# Autodesk Inventor assembly: MARS Micromouse Box
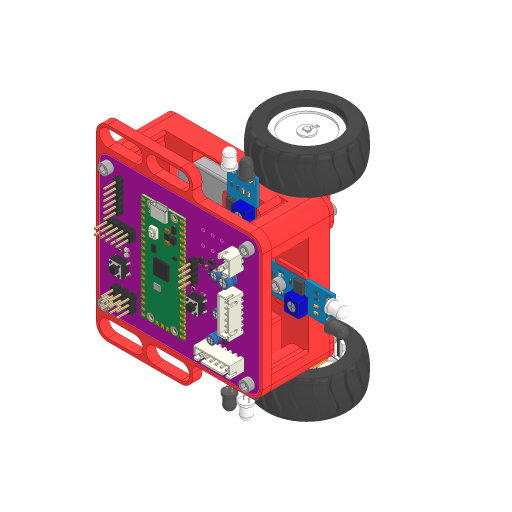
[picture p0: Inventor's stored thumbnail of the model, 512x512]
Saved by Autodesk Inventor 2024 (Build 280153000, 153)
## iProperties
Created: 2026-07-12
Part Number: MARS Micromouse Box
Document SubType Name: Assembly
Designer: Binara
Title: MARS Micromouse.step
Sending System: Autodesk Translation Framework v15.8.0.0
Preprocessor: ST-DEVELOPER v20.1
## Documents named in this file (12)
- Z:\Robotics\MARS\Micromouse Robot\starter-micromouse\CAD\MARS Micromouse\MARS Micromouse.iam
- Z:\Robotics\MARS\Micromouse Robot\starter-micromouse\CAD\MARS Micromouse\MARS_Micromouse_PCB v1.iam
- Z:\Robotics\MARS\Micromouse Robot\starter-micromouse\CAD\MARS Micromouse\Top Plate.ipt
- Z:\Robotics\MARS\Micromouse Robot\starter-micromouse\CAD\MARS Micromouse\Base Plate.ipt
- Z:\Robotics\MARS\Micromouse Robot\starter-micromouse\CAD\MARS Micromouse\IR_Sensor_YL63 v1.ipt
- Z:\Robotics\MARS\Micromouse Robot\starter-micromouse\CAD\MARS Micromouse\N20 Mini Micro Metall Gear Motor v1.ipt
- Z:\Robotics\MARS\Micromouse Robot\starter-micromouse\CAD\MARS Micromouse\RC wheel v1.iam
- Z:\Robotics\MARS\Micromouse Robot\starter-micromouse\CAD\MARS Micromouse\Motor Clamp.ipt
- Z:\Robotics\MARS\Micromouse Robot\starter-micromouse\CAD\MARS Micromouse\Caster Ball Extension.ipt
- Z:\Robotics\MARS\Micromouse Robot\starter-micromouse\CAD\MARS Micromouse\Caster Ball v3.ipt
- Z:\Robotics\MARS\Micromouse Robot\starter-micromouse\CAD\MARS Micromouse\New Battery.ipt
- Z:\Robotics\Inventor\Hardware\M3 x 8 screw\M3 x 8 screw.ipt
## Components (30 placed, 11 different names)
1. MARS_Micromouse_PCB v1:1 [sub-assembly] — Rigid:2, Cylindrical:1, Cylindrical:2, Rigid:3
2. Top Plate:1
3. Base Plate:1
4. IR_Sensor_YL63 v1:1 — Rotational:8
5. IR_Sensor_YL63 v1:2 — Rotational:9
6. IR_Sensor_YL63 v1:3 — Rotational:10
7. N20 Mini Micro Metall Gear Motor v1:1
8. N20 Mini Micro Metall Gear Motor v1:2
9. RC wheel v1:1 [sub-assembly]
10. RC wheel v1:2 [sub-assembly]
11. Motor Clamp:1 — Rotational:2, Rotational:3
12. Motor Clamp:2 — Rotational:4, Rotational:5
13. Caster Ball Extension:1 — Rotational:6, Rotational:7
14. Caster Ball v3:1 — Rigid:1, Rotational:1
15. New Battery:1
16. M3 x 8 screw:1 — Rotational:8
17. M3 x 8 screw:2 — Rigid:2
18. M3 x 8 screw:3 — Cylindrical:2
19. M3 x 8 screw:4 — Rigid:3
20. M3 x 8 screw:5 — Cylindrical:1
21. M3 x 8 screw:6 — Rotational:7
22. M3 x 8 screw:7 — Rotational:2
23. M3 x 8 screw:8 — Rotational:3
24. M3 x 8 screw:9 — Rotational:4
25. M3 x 8 screw:10 — Rotational:5
26. M3 x 8 screw:11 — Rotational:6
27. M3 x 8 screw:12 — Rigid:1
28. M3 x 8 screw:13 — Rotational:1
29. M3 x 8 screw:14 — Rotational:9
30. M3 x 8 screw:15 — Rotational:10
## Relationships (15: RevoluteJoint 10, WeldJoint 3, CylindricalJoint 2)
- Rigid:1 [WeldJoint]: Caster Ball v3:1 ↔ M3 x 8 screw:12
- Rotational:1 [RevoluteJoint]: Caster Ball v3:1 ↔ M3 x 8 screw:13
- Rotational:2 [RevoluteJoint]: Motor Clamp:1 ↔ M3 x 8 screw:7
- Rotational:3 [RevoluteJoint]: Motor Clamp:1 ↔ M3 x 8 screw:8
- Rotational:4 [RevoluteJoint]: Motor Clamp:2 ↔ M3 x 8 screw:9
- Rotational:5 [RevoluteJoint]: Motor Clamp:2 ↔ M3 x 8 screw:10
- Rotational:6 [RevoluteJoint]: Caster Ball Extension:1 ↔ M3 x 8 screw:11
- Rotational:7 [RevoluteJoint]: Caster Ball Extension:1 ↔ M3 x 8 screw:6
- Rigid:2 [WeldJoint]: MARS_Micromouse_PCB v1:1 ↔ M3 x 8 screw:2
- Cylindrical:1: MARS_Micromouse_PCB v1:1 ↔ M3 x 8 screw:5
- Cylindrical:2: MARS_Micromouse_PCB v1:1 ↔ M3 x 8 screw:3
- Rigid:3 [WeldJoint]: MARS_Micromouse_PCB v1:1 ↔ M3 x 8 screw:4
- Rotational:8 [RevoluteJoint]: IR_Sensor_YL63 v1:1 ↔ M3 x 8 screw:1
- Rotational:9 [RevoluteJoint]: IR_Sensor_YL63 v1:2 ↔ M3 x 8 screw:14
- Rotational:10 [RevoluteJoint]: IR_Sensor_YL63 v1:3 ↔ M3 x 8 screw:15
